# Autodesk Inventor assembly: erp42_2
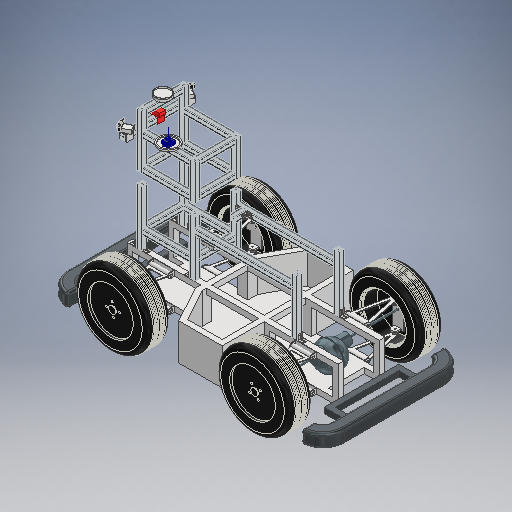
[picture p0: Inventor's stored thumbnail of the model, 512x512]
Saved by Autodesk Inventor 2025.2 (Build 292293000, 293)
## iProperties
Created: 2024-02-06
Part Number: erp42_2
Document SubType Name: Assembly
Designer: ps737
Author: ps737
## Documents named in this file (29)
- C:\Users\jbhma\OneDrive\Desktop\2025_ACCA\2024 ERP42\erp42_2.iam
- C:\Users\jbhma\OneDrive\Desktop\2025_ACCA\2024 ERP42\body.ipt
- C:\Users\jbhma\OneDrive\Desktop\2025_ACCA\2024 ERP42\bumper.ipt
- C:\Users\jbhma\OneDrive\Desktop\2025_ACCA\2024 ERP42\body_braket.ipt
- C:\Users\jbhma\OneDrive\Desktop\2025_ACCA\2024 ERP42\link.ipt
- C:\Users\jbhma\OneDrive\Desktop\2025_ACCA\2024 ERP42\wheel.ipt
- C:\Users\jbhma\OneDrive\Desktop\2025_ACCA\2024 ERP42\wheel_bolt.ipt
- C:\Users\jbhma\OneDrive\Desktop\2025_ACCA\2024 ERP42\프로파일\34.ipt
- C:\Users\jbhma\OneDrive\Desktop\2025_ACCA\2024 ERP42\프로파일\40.5.ipt
- C:\Users\jbhma\OneDrive\Desktop\2025_ACCA\2024 ERP42\L자 브라켓.ipt
- C:\Users\jbhma\OneDrive\Desktop\2025_ACCA\2024 ERP42\wheel_braket_13.ipt
- C:\Users\jbhma\OneDrive\Desktop\2025_ACCA\2024 ERP42\wheel_braket_24.ipt
- C:\Users\jbhma\OneDrive\Desktop\2025_ACCA\2024 ERP42\base_link.ipt
- base_link.ipt
- C:\Users\jbhma\OneDrive\Desktop\2025_ACCA\2024 ERP42\프로파일\8.ipt
- C:\Users\jbhma\OneDrive\Desktop\2025_ACCA\2024 ERP42\프로파일\26.ipt
- C:\Users\jbhma\OneDrive\Desktop\2025_ACCA\2024 ERP42\프로파일\39.ipt
- C:\Users\jbhma\OneDrive\Desktop\2025_ACCA\2024 ERP42\프로파일\70.5.ipt
- C:\Users\jbhma\OneDrive\Desktop\2025_ACCA\2024 ERP42\lidar_case.ipt
- C:\Users\jbhma\OneDrive\Desktop\2025_ACCA\2024 ERP42\86-0138 REV 2, ENVELOPE, VLP-32C M12M.iam
- C:\Users\jbhma\OneDrive\Desktop\2025_ACCA\2024 ERP42\gps_case.ipt
- C:\Users\jbhma\OneDrive\Desktop\2025_ACCA\2024 ERP42\UBLOX_ANN-MB-00_GNSS_ANTENNA.ipt
- C:\Users\jbhma\OneDrive\Desktop\2025_ACCA\2024 ERP42\프로파일\50.ipt
- C:\Users\jbhma\OneDrive\Desktop\2025_ACCA\2024 ERP42\camera_case_front.ipt
- C:\Users\jbhma\OneDrive\Desktop\2025_ACCA\2024 ERP42\camera_case_left.ipt
- C:\Users\jbhma\OneDrive\Desktop\2025_ACCA\2024 ERP42\camera_case_right.ipt
- C:\Users\jbhma\OneDrive\Desktop\2025_ACCA\2024 ERP42\camera.ipt
- C:\Users\jbhma\OneDrive\Desktop\2025_ACCA\2024 ERP42\imu_case.ipt
- C:\Users\jbhma\OneDrive\Desktop\2025_ACCA\2024 ERP42\MTi 600-series STEP files\MTi-600 DEV assembly.iam
## Components (88 placed, 27 different names)
1. body:1 — 메이트:1, 메이트:2, 메이트:3, 메이트:4, 메이트:5, 메이트:6, 메이트:9, 메이트:12, 메이트:60, 메이트:61, 플러쉬:1, 플러쉬:3, 플러쉬:4, 메이트:62, 메이트:64, 메이트:65, 플러쉬:6, 플러쉬:7, 플러쉬:8, 메이트:77, 메이트:78, 메이트:79, 플러쉬:9, 플러쉬:10, 플러쉬:11, 메이트:107, 메이트:108, 플러쉬:21, 플러쉬:22, 메이트:109, 메이트:110, 메이트:124, 플러쉬:28, 각도:18, 플러쉬:29, 각도:19, 플러쉬:31, 플러쉬:32, 플러쉬:33, 메이트:152, 메이트:153, 메이트:154, 각도:20, 각도:21, 각도:22, 각도:23, 메이트:192, 플러쉬:34, 메이트:194, 플러쉬:35, 메이트:196, 플러쉬:36, 메이트:198, 플러쉬:37, 메이트:200, 플러쉬:38, 메이트:202, 플러쉬:39, 메이트:204, 메이트:206, 플러쉬:41, 메이트:209, 플러쉬:42, 메이트:241, 메이트:242, 메이트:243, 플러쉬:60, 메이트:244, 플러쉬:61, 메이트:245, 플러쉬:62, 메이트:252, 메이트:255
2. bumper:1 — 메이트:1, 메이트:2, 플러쉬:6, 플러쉬:10
3. bumper:2 — 메이트:3, 메이트:4, 플러쉬:7, 플러쉬:11, 플러쉬:58
4. body_braket:5 — 메이트:5, 플러쉬:32, 메이트:145, 메이트:151, 메이트:153
5. body_braket:7 — 메이트:6, 메이트:133, 메이트:134, 플러쉬:29, 플러쉬:30
6. body_braket:10 — 메이트:9, 플러쉬:3, 메이트:65, 메이트:144, 메이트:150
7. body_braket:12 — 메이트:12, 플러쉬:1, 메이트:62, 메이트:135, 메이트:136, 플러쉬:30, 플러쉬:40
8. body_braket:15 — 메이트:61, 메이트:140, 메이트:143, 플러쉬:31, 메이트:154
9. body_braket:16 — 메이트:60, 플러쉬:4, 메이트:64, 메이트:141, 메이트:142
10. body_braket:17 — 메이트:79, 플러쉬:33, 메이트:146, 메이트:148, 메이트:152
11. body_braket:18 — 메이트:77, 메이트:78, 플러쉬:9, 메이트:147, 메이트:149
12. 40.5:1 — 메이트:107, 플러쉬:21, 메이트:109, 메이트:201, 메이트:225, 플러쉬:52, 플러쉬:59, 플러쉬:110
13. 40.5:2 — 메이트:108, 플러쉬:22, 메이트:110, 메이트:205, 플러쉬:42, 메이트:224, 플러쉬:51, 플러쉬:109
14. 40.5:3 — 메이트:124, 플러쉬:28, 메이트:203, 메이트:214, 메이트:227, 플러쉬:53, 메이트:249, 플러쉬:66, 메이트:274, 플러쉬:107
15. link:19 — 메이트:129, 메이트:130, 메이트:133, 메이트:134
16. wheel_braket_13:1 — 메이트:131, 메이트:132, 각도:19, 메이트:137, 메이트:139, 메이트:179, 각도:23, 메이트:185
17. wheel_bolt:11 — 메이트:129, 메이트:130, 메이트:131, 메이트:132
18. link:20 — 메이트:135, 메이트:136, 각도:18, 메이트:138, 메이트:240
19. wheel_bolt:12 — 메이트:137, 메이트:138, 메이트:139, 메이트:240
20. link:21 — 메이트:141, 메이트:142, 메이트:175, 메이트:177
21. link:22 — 메이트:140, 메이트:143, 메이트:176, 메이트:178, 메이트:184
22. link:23 — 메이트:146, 메이트:148, 메이트:172, 메이트:174
23. link:24 — 메이트:147, 메이트:149, 메이트:171, 메이트:173
24. link:25 — 메이트:144, 메이트:150, 메이트:167, 메이트:168
25. link:26 — 메이트:145, 메이트:151, 메이트:169, 메이트:170
26. wheel:1 — 메이트:186, 메이트:187
27. wheel:2 — 메이트:179, 메이트:185
28. wheel:3 — 메이트:190, 메이트:191
29. wheel:4 — 메이트:188, 메이트:189, 메이트:208, 메이트:210
30. wheel_braket_13:2 — 메이트:155, 메이트:156, 메이트:161, 메이트:162, 각도:21, 메이트:190, 메이트:191
31. wheel_braket_24:1 — 메이트:180, 메이트:181, 메이트:182, 메이트:183, 각도:20, 메이트:186, 메이트:187
32. wheel_braket_24:2 — 메이트:157, 메이트:158, 메이트:163, 메이트:164, 각도:22, 메이트:188, 메이트:189
33. wheel_bolt:13 — 메이트:158, 메이트:163, 메이트:172, 메이트:174
34. wheel_bolt:14 — 메이트:155, 메이트:161, 메이트:169, 메이트:170
35. wheel_bolt:15 — 메이트:157, 메이트:164, 메이트:171, 메이트:173
36. wheel_bolt:16 — 메이트:156, 메이트:162, 메이트:167, 메이트:168
37. wheel_bolt:17 — 메이트:175, 메이트:177, 메이트:180, 메이트:181, 메이트:183
38. wheel_bolt:18 — 메이트:176, 메이트:178, 메이트:182, 메이트:184
39. L자 브라켓:1 — 메이트:194, 플러쉬:35
40. L자 브라켓:2 — 메이트:192, 플러쉬:34
41. L자 브라켓:3 — 메이트:196, 플러쉬:36
42. L자 브라켓:4 — 메이트:198, 플러쉬:37
43. L자 브라켓:5 — 메이트:202, 메이트:203, 플러쉬:39
44. L자 브라켓:6 — 메이트:200, 메이트:201, 플러쉬:38, 플러쉬:59
45. L자 브라켓:7 — 메이트:204, 메이트:205, 플러쉬:40
46. L자 브라켓:8 — 메이트:206, 플러쉬:41, 메이트:250
47. base_link:1 — 메이트:208, 메이트:209, 메이트:210
48. 8:1 — 메이트:214, 메이트:217, 메이트:218
49. L자 브라켓:9 — 메이트:217
50. L자 브라켓:10 — 메이트:218
51. L자 브라켓:13
52. L자 브라켓:14 — 메이트:224, 플러쉬:51, 메이트:275
53. L자 브라켓:15 — 메이트:225, 플러쉬:52, 메이트:276
54. L자 브라켓:17 — 메이트:227, 플러쉬:53
55. 40.5:4 — 메이트:243, 플러쉬:60, 메이트:246, 플러쉬:64, 메이트:251, 메이트:253, 플러쉬:67, 플러쉬:105, 플러쉬:106
56. 40.5:5 — 메이트:245, 플러쉬:62, 메이트:247, 플러쉬:63, 메이트:254, 플러쉬:68
57. 40.5:6 — 메이트:244, 플러쉬:61, 메이트:248, 플러쉬:65, 메이트:250, 메이트:251, 메이트:252, 메이트:273, 플러쉬:108, 플러쉬:122
58. 26:1 — 메이트:246, 메이트:247, 플러쉬:63, 플러쉬:64, 플러쉬:69, 플러쉬:70, 플러쉬:71, 메이트:255
59. 26:2 — 메이트:248, 메이트:249, 플러쉬:65, 플러쉬:66, 플러쉬:71, 메이트:303, 플러쉬:123
60. 34:1 — 메이트:253, 플러쉬:67, 플러쉬:70
61. 34:2 — 메이트:254, 플러쉬:68, 플러쉬:69
62. 39:3 — 메이트:260, 메이트:262, 플러쉬:72, 플러쉬:75, 플러쉬:76, 플러쉬:86, 메이트:268, 플러쉬:95, 플러쉬:96, 플러쉬:105, 플러쉬:106, 메이트:282
63. 39:4 — 메이트:261, 메이트:263, 플러쉬:73, 플러쉬:74, 플러쉬:77, 플러쉬:87, 메이트:270, 플러쉬:97, 플러쉬:98, 메이트:299, 플러쉬:120
64. 26:3 — 메이트:264, 메이트:267, 플러쉬:92, 플러쉬:93, 플러쉬:94
65. 26:4 — 메이트:260, 메이트:261, 플러쉬:72, 플러쉬:73, 플러쉬:74, 플러쉬:75, 각도:24, 각도:25, 플러쉬:111, 메이트:298
66. 26:5 — 메이트:262, 메이트:263, 플러쉬:76, 플러쉬:77, 플러쉬:86, 플러쉬:87
67. 26:6 — 메이트:265, 플러쉬:88, 플러쉬:89, 플러쉬:90, 플러쉬:91, 플러쉬:119
68. 26:7 — 플러쉬:90, 메이트:267, 플러쉬:91, 플러쉬:93, 플러쉬:99, 플러쉬:100, 메이트:271, 플러쉬:102, 플러쉬:103
69. 26:8 — 메이트:264, 메이트:265, 플러쉬:88, 플러쉬:89, 플러쉬:92, 플러쉬:94, 메이트:269, 메이트:272, 플러쉬:101, 플러쉬:104
70. 34:4 — 메이트:268, 메이트:269, 플러쉬:95, 플러쉬:96
71. 34:5 — 메이트:270, 플러쉬:97, 플러쉬:98, 플러쉬:99, 플러쉬:100
72. 34:6 — 메이트:271, 플러쉬:102, 플러쉬:103, 플러쉬:121
73. 34:7 — 메이트:272, 플러쉬:101, 플러쉬:104, 메이트:285, 플러쉬:112
74. 70.5:2 — 메이트:274, 플러쉬:107, 플러쉬:109, 메이트:276
75. 70.5:3 — 메이트:273, 플러쉬:108, 플러쉬:110, 메이트:275
76. lidar_case:1 — 각도:24, 메이트:280, 메이트:281, 메이트:282, 메이트:298
77. 86-0138 REV 2, ENVELOPE, VLP-32C M12M:1 [sub-assembly] — 메이트:280, 메이트:281, 각도:25, 플러쉬:111
78. gps_case:1 — 메이트:284, 메이트:285, 플러쉬:112
79. UBLOX_ANN-MB-00_GNSS_ANTENNA:1 — 메이트:284, 플러쉬:119
80. 50:1 — 메이트:292, 메이트:293, 메이트:294, 메이트:295, 메이트:296, 메이트:297, 플러쉬:116, 플러쉬:117, 플러쉬:118, 메이트:299, 플러쉬:120, 플러쉬:121
81. camera_case_front:1 — 메이트:290, 메이트:291, 플러쉬:115, 메이트:292, 메이트:293, 플러쉬:116
82. camera_case_left:1 — 메이트:286, 메이트:287, 플러쉬:113, 메이트:294, 메이트:295, 플러쉬:118
83. camera_case_right:1 — 메이트:288, 메이트:289, 플러쉬:114, 메이트:296, 메이트:297, 플러쉬:117
84. camera:1 — 메이트:288, 메이트:289, 플러쉬:114
85. camera:2 — 메이트:286, 메이트:287, 플러쉬:113
86. camera:3 — 메이트:290, 메이트:291, 플러쉬:115
87. imu_case:1 — 메이트:303, 플러쉬:122, 플러쉬:123
88. MTi-600 DEV assembly:1 [sub-assembly]
## Relationships (252: Mate 156, Flush 87, Angle 9)
- 메이트:1 [Mate]: body:1 ↔ bumper:1
- 메이트:2 [Mate]: body:1 ↔ bumper:1
- 메이트:3 [Mate]: body:1 ↔ bumper:2
- 메이트:4 [Mate]: body:1 ↔ bumper:2
- 메이트:5 [Mate]: body:1 ↔ body_braket:5
- 메이트:6 [Mate]: body:1 ↔ body_braket:7
- 메이트:9 [Mate]: body:1 ↔ body_braket:10
- 메이트:12 [Mate]: body:1 ↔ body_braket:12
- 메이트:60 [Mate]: body:1 ↔ body_braket:16
- 메이트:61 [Mate]: body:1 ↔ body_braket:15
- 플러쉬:1 [Flush]: body:1 ↔ body_braket:12
- 플러쉬:3 [Flush]: body:1 ↔ body_braket:10
- 플러쉬:4 [Flush]: body:1 ↔ body_braket:16
- 메이트:62 [Mate] (230 mm): body:1 ↔ body_braket:12
- 메이트:64 [Mate] (190 mm): body:1 ↔ body_braket:16
- 메이트:65 [Mate] (190 mm): body:1 ↔ body_braket:10
- 플러쉬:6 [Flush] (-25 mm): body:1 ↔ bumper:1
- 플러쉬:7 [Flush] (-25 mm): body:1 ↔ bumper:2
- 플러쉬:8 [Flush] (105 mm): body:1
- 메이트:77 [Mate]: body:1 ↔ body_braket:18
- 메이트:78 [Mate] (230 mm): body:1 ↔ body_braket:18
- 메이트:79 [Mate]: body:1 ↔ body_braket:17
- 플러쉬:9 [Flush]: body:1 ↔ body_braket:18
- 플러쉬:10 [Flush] (100 mm): body:1 ↔ bumper:1
- 플러쉬:11 [Flush] (100 mm): body:1 ↔ bumper:2
- 메이트:107 [Mate]: body:1 ↔ 40.5:1
- 메이트:108 [Mate]: body:1 ↔ 40.5:2
- 플러쉬:21 [Flush]: body:1 ↔ 40.5:1
- 플러쉬:22 [Flush]: body:1 ↔ 40.5:2
- 메이트:109 [Mate] (200 mm): body:1 ↔ 40.5:1
- 메이트:110 [Mate] (200 mm): body:1 ↔ 40.5:2
- 메이트:124 [Mate]: body:1 ↔ 40.5:3
- 플러쉬:28 [Flush]: body:1 ↔ 40.5:3
- 메이트:129 [Mate]: link:19 ↔ wheel_bolt:11
- 메이트:130 [Mate]: link:19 ↔ wheel_bolt:11
- 메이트:131 [Mate]: wheel_braket_13:1 ↔ wheel_bolt:11
- 메이트:132 [Mate]: wheel_braket_13:1 ↔ wheel_bolt:11
- 메이트:133 [Mate]: body_braket:7 ↔ link:19
- 메이트:134 [Mate]: body_braket:7 ↔ link:19
- 메이트:135 [Mate]: body_braket:12 ↔ link:20
- 메이트:136 [Mate]: body_braket:12 ↔ link:20
- 각도:18 [Angle] (0 deg): body:1 ↔ link:20
- 플러쉬:29 [Flush]: body:1 ↔ body_braket:7
- 각도:19 [Angle] (180 deg): body:1 ↔ wheel_braket_13:1
- 플러쉬:30 [Flush]: body_braket:7 ↔ body_braket:12
- 메이트:137 [Mate]: wheel_braket_13:1 ↔ wheel_bolt:12
- 메이트:138 [Mate]: link:20 ↔ wheel_bolt:12
- 메이트:139 [Mate]: wheel_braket_13:1 ↔ wheel_bolt:12
- 메이트:140 [Mate]: body_braket:15 ↔ link:22
- 메이트:141 [Mate]: body_braket:16 ↔ link:21
- 메이트:142 [Mate]: body_braket:16 ↔ link:21
- 메이트:143 [Mate]: body_braket:15 ↔ link:22
- 플러쉬:31 [Flush]: body:1 ↔ body_braket:15
- 플러쉬:32 [Flush]: body:1 ↔ body_braket:5
- 플러쉬:33 [Flush]: body:1 ↔ body_braket:17
- 메이트:144 [Mate]: body_braket:10 ↔ link:25
- 메이트:145 [Mate]: body_braket:5 ↔ link:26
- 메이트:146 [Mate]: body_braket:17 ↔ link:23
- 메이트:147 [Mate]: body_braket:18 ↔ link:24
- 메이트:148 [Mate]: body_braket:17 ↔ link:23
- 메이트:149 [Mate]: body_braket:18 ↔ link:24
- 메이트:150 [Mate]: body_braket:10 ↔ link:25
- 메이트:151 [Mate]: body_braket:5 ↔ link:26
- 메이트:152 [Mate] (230 mm): body:1 ↔ body_braket:17
- 메이트:153 [Mate] (190 mm): body:1 ↔ body_braket:5
- 메이트:154 [Mate] (190 mm): body:1 ↔ body_braket:15
- 메이트:155 [Mate]: wheel_braket_13:2 ↔ wheel_bolt:14
- 메이트:156 [Mate]: wheel_braket_13:2 ↔ wheel_bolt:16
- 메이트:157 [Mate]: wheel_braket_24:2 ↔ wheel_bolt:15
- 메이트:158 [Mate]: wheel_braket_24:2 ↔ wheel_bolt:13
- 메이트:161 [Mate]: wheel_braket_13:2 ↔ wheel_bolt:14
- 메이트:162 [Mate]: wheel_braket_13:2 ↔ wheel_bolt:16
- 메이트:163 [Mate]: wheel_braket_24:2 ↔ wheel_bolt:13
- 메이트:164 [Mate]: wheel_braket_24:2 ↔ wheel_bolt:15
- 메이트:167 [Mate]: link:25 ↔ wheel_bolt:16
- 메이트:168 [Mate]: link:25 ↔ wheel_bolt:16
- 메이트:169 [Mate]: link:26 ↔ wheel_bolt:14
- 메이트:170 [Mate]: link:26 ↔ wheel_bolt:14
- 메이트:171 [Mate]: link:24 ↔ wheel_bolt:15
- 메이트:172 [Mate]: link:23 ↔ wheel_bolt:13
- 메이트:173 [Mate]: link:24 ↔ wheel_bolt:15
- 메이트:174 [Mate]: link:23 ↔ wheel_bolt:13
- 메이트:175 [Mate]: link:21 ↔ wheel_bolt:17
- 메이트:176 [Mate]: link:22 ↔ wheel_bolt:18
- 메이트:177 [Mate]: link:21 ↔ wheel_bolt:17
- 메이트:178 [Mate]: link:22 ↔ wheel_bolt:18
- 메이트:179 [Mate]: wheel_braket_13:1 ↔ wheel:2
- 메이트:180 [Mate]: wheel_braket_24:1 ↔ wheel_bolt:17
- 메이트:181 [Mate]: wheel_braket_24:1 ↔ wheel_bolt:17
- 메이트:182 [Mate]: wheel_braket_24:1 ↔ wheel_bolt:18
- 메이트:183 [Mate]: wheel_braket_24:1 ↔ wheel_bolt:17
- 메이트:184 [Mate]: link:22 ↔ wheel_bolt:18
- 각도:20 [Angle] (180 deg): body:1 ↔ wheel_braket_24:1
- 각도:21 [Angle] (180 deg): body:1 ↔ wheel_braket_13:2
- 각도:22 [Angle] (180 deg): body:1 ↔ wheel_braket_24:2
- 각도:23 [Angle] (180 deg): body:1 ↔ wheel_braket_13:1
- 메이트:185 [Mate]: wheel_braket_13:1 ↔ wheel:2
- 메이트:186 [Mate]: wheel:1 ↔ wheel_braket_24:1
- 메이트:187 [Mate]: wheel:1 ↔ wheel_braket_24:1
- 메이트:188 [Mate]: wheel:4 ↔ wheel_braket_24:2
- 메이트:189 [Mate]: wheel:4 ↔ wheel_braket_24:2
- 메이트:190 [Mate]: wheel:3 ↔ wheel_braket_13:2
- 메이트:191 [Mate]: wheel:3 ↔ wheel_braket_13:2
- 메이트:192 [Mate]: body:1 ↔ L자 브라켓:2
- 플러쉬:34 [Flush] (2.5 mm): body:1 ↔ L자 브라켓:2
- 메이트:194 [Mate]: body:1 ↔ L자 브라켓:1
- 플러쉬:35 [Flush] (2.5 mm): body:1 ↔ L자 브라켓:1
- 메이트:196 [Mate]: body:1 ↔ L자 브라켓:3
- 플러쉬:36 [Flush] (2.2 mm): body:1 ↔ L자 브라켓:3
- 메이트:198 [Mate]: body:1 ↔ L자 브라켓:4
- 플러쉬:37 [Flush] (2.5 mm): body:1 ↔ L자 브라켓:4
- 메이트:200 [Mate]: body:1 ↔ L자 브라켓:6
- 메이트:201 [Mate]: 40.5:1 ↔ L자 브라켓:6
- 플러쉬:38 [Flush] (2.5 mm): body:1 ↔ L자 브라켓:6
- 메이트:202 [Mate]: body:1 ↔ L자 브라켓:5
- 메이트:203 [Mate]: 40.5:3 ↔ L자 브라켓:5
- 플러쉬:39 [Flush] (2.5 mm): body:1 ↔ L자 브라켓:5
- 메이트:204 [Mate]: body:1 ↔ L자 브라켓:7
- 메이트:205 [Mate]: 40.5:2 ↔ L자 브라켓:7
- 플러쉬:40 [Flush] (2.5 mm): body_braket:12 ↔ L자 브라켓:7
- 메이트:206 [Mate]: body:1 ↔ L자 브라켓:8
- 플러쉬:41 [Flush] (2.5 mm): body:1 ↔ L자 브라켓:8
- 메이트:208 [Mate]: wheel:4 ↔ base_link:1
- 메이트:209 [Mate]: body:1 ↔ base_link:1
- 메이트:210 [Mate]: wheel:4 ↔ base_link:1
- 플러쉬:42 [Flush]: body:1 ↔ 40.5:2
- 메이트:214 [Mate] (40 mm): 40.5:3 ↔ 8:1
- 메이트:217 [Mate]: 8:1 ↔ L자 브라켓:9
- 메이트:218 [Mate]: 8:1 ↔ L자 브라켓:10
- 메이트:224 [Mate]: 40.5:2 ↔ L자 브라켓:14
- 플러쉬:51 [Flush] (2.5 mm): 40.5:2 ↔ L자 브라켓:14
- 메이트:225 [Mate]: 40.5:1 ↔ L자 브라켓:15
- 플러쉬:52 [Flush] (2.5 mm): 40.5:1 ↔ L자 브라켓:15
- 메이트:227 [Mate]: 40.5:3 ↔ L자 브라켓:17
- 플러쉬:53 [Flush] (2.5 mm): 40.5:3 ↔ L자 브라켓:17
- 메이트:240 [Mate]: link:20 ↔ wheel_bolt:12
- 메이트:241 [Mate] (-170 mm): body:1
- 메이트:242 [Mate] (105 mm): body:1
- 플러쉬:58 [Flush] (-990 mm): bumper:2
- 플러쉬:59 [Flush] (2.5 mm): 40.5:1 ↔ L자 브라켓:6
- 메이트:243 [Mate]: body:1 ↔ 40.5:4
- 플러쉬:60 [Flush]: body:1 ↔ 40.5:4
- 메이트:244 [Mate]: body:1 ↔ 40.5:6
- 플러쉬:61 [Flush]: body:1 ↔ 40.5:6
- 메이트:245 [Mate]: body:1 ↔ 40.5:5
- 플러쉬:62 [Flush]: body:1 ↔ 40.5:5
- 메이트:246 [Mate]: 40.5:4 ↔ 26:1
- 메이트:247 [Mate]: 40.5:5 ↔ 26:1
- 플러쉬:63 [Flush]: 40.5:5 ↔ 26:1
- 플러쉬:64 [Flush]: 40.5:4 ↔ 26:1
- 메이트:248 [Mate]: 40.5:6 ↔ 26:2
- 메이트:249 [Mate]: 40.5:3 ↔ 26:2
- 플러쉬:65 [Flush]: 40.5:6 ↔ 26:2
- 플러쉬:66 [Flush]: 40.5:3 ↔ 26:2
- 메이트:250 [Mate]: L자 브라켓:8 ↔ 40.5:6
- 메이트:251 [Mate] (340 mm): 40.5:4 ↔ 40.5:6
- 메이트:252 [Mate] (45 mm): body:1 ↔ 40.5:6
- 메이트:253 [Mate]: 40.5:4 ↔ 34:1
- 메이트:254 [Mate]: 40.5:5 ↔ 34:2
- 플러쉬:67 [Flush]: 40.5:4 ↔ 34:1
- 플러쉬:68 [Flush]: 40.5:5 ↔ 34:2
- 플러쉬:69 [Flush]: 26:1 ↔ 34:2
- 플러쉬:70 [Flush]: 26:1 ↔ 34:1
- 플러쉬:71 [Flush]: 26:1 ↔ 26:2
- 메이트:255 [Mate] (100 mm): body:1 ↔ 26:1
- 메이트:260 [Mate]: 39:3 ↔ 26:4
- 메이트:261 [Mate]: 39:4 ↔ 26:4
- 메이트:262 [Mate]: 39:3 ↔ 26:5
- 메이트:263 [Mate]: 39:4 ↔ 26:5
- 플러쉬:72 [Flush]: 39:3 ↔ 26:4
- 플러쉬:73 [Flush]: 39:4 ↔ 26:4
- 플러쉬:74 [Flush]: 39:4 ↔ 26:4
- 플러쉬:75 [Flush]: 39:3 ↔ 26:4
- 플러쉬:76 [Flush]: 39:3 ↔ 26:5
- 플러쉬:77 [Flush]: 39:4 ↔ 26:5
- 플러쉬:86 [Flush]: 39:3 ↔ 26:5
- 플러쉬:87 [Flush]: 39:4 ↔ 26:5
- 메이트:264 [Mate]: 26:3 ↔ 26:8
- 메이트:265 [Mate]: 26:6 ↔ 26:8
- 플러쉬:88 [Flush]: 26:6 ↔ 26:8
- 플러쉬:89 [Flush]: 26:6 ↔ 26:8
- 플러쉬:90 [Flush]: 26:6 ↔ 26:7
- 메이트:267 [Mate]: 26:3 ↔ 26:7
- 플러쉬:91 [Flush]: 26:6 ↔ 26:7
- 플러쉬:92 [Flush]: 26:3 ↔ 26:8
- 플러쉬:93 [Flush]: 26:3 ↔ 26:7
- 플러쉬:94 [Flush]: 26:3 ↔ 26:8
- 메이트:268 [Mate]: 39:3 ↔ 34:4
- 메이트:269 [Mate]: 26:8 ↔ 34:4
- 플러쉬:95 [Flush]: 39:3 ↔ 34:4
- 플러쉬:96 [Flush]: 39:3 ↔ 34:4
- 메이트:270 [Mate]: 39:4 ↔ 34:5
- 플러쉬:97 [Flush]: 39:4 ↔ 34:5
- 플러쉬:98 [Flush]: 39:4 ↔ 34:5
- 플러쉬:99 [Flush]: 26:7 ↔ 34:5
- 플러쉬:100 [Flush]: 26:7 ↔ 34:5
- 메이트:271 [Mate]: 26:7 ↔ 34:6
- 메이트:272 [Mate]: 26:8 ↔ 34:7
- 플러쉬:101 [Flush]: 26:8 ↔ 34:7
- 플러쉬:102 [Flush]: 26:7 ↔ 34:6
- 플러쉬:103 [Flush]: 26:7 ↔ 34:6
- 플러쉬:104 [Flush]: 26:8 ↔ 34:7
- 플러쉬:105 [Flush]: 40.5:4 ↔ 39:3
- 플러쉬:106 [Flush]: 40.5:4 ↔ 39:3
- 메이트:273 [Mate]: 40.5:6 ↔ 70.5:3
- 메이트:274 [Mate]: 40.5:3 ↔ 70.5:2
- 플러쉬:107 [Flush]: 40.5:3 ↔ 70.5:2
- 플러쉬:108 [Flush]: 40.5:6 ↔ 70.5:3
- 플러쉬:109 [Flush] (73 mm): 40.5:2 ↔ 70.5:2
- 플러쉬:110 [Flush] (73 mm): 40.5:1 ↔ 70.5:3
- 메이트:275 [Mate]: L자 브라켓:14 ↔ 70.5:3
- 메이트:276 [Mate]: L자 브라켓:15 ↔ 70.5:2
- 각도:24 [Angle] (90 deg): 26:4 ↔ lidar_case:1
- 메이트:280 [Mate]: lidar_case:1 ↔ 86-0138 REV 2, ENVELOPE, VLP-32C M12M:1
- 메이트:281 [Mate]: lidar_case:1 ↔ 86-0138 REV 2, ENVELOPE, VLP-32C M12M:1
- 메이트:282 [Mate] (137 mm): 39:3 ↔ lidar_case:1
- 각도:25 [Angle] (180 deg): 26:4 ↔ 86-0138 REV 2, ENVELOPE, VLP-32C M12M:1
- 플러쉬:111 [Flush] (-39.055 mm): 26:4 ↔ 86-0138 REV 2, ENVELOPE, VLP-32C M12M:1
- [Mate]: gps_case:1 ↔ UBLOX_ANN-MB-00_GNSS_ANTENNA:1
- [Angle] (270 deg): gps_case:1 ↔ UBLOX_ANN-MB-00_GNSS_ANTENNA:1
- 메이트:284 [Mate]: gps_case:1 ↔ UBLOX_ANN-MB-00_GNSS_ANTENNA:1
- 메이트:285 [Mate]: 34:7 ↔ gps_case:1
- 플러쉬:112 [Flush] (25 mm): 34:7 ↔ gps_case:1
- 메이트:286 [Mate]: camera_case_left:1 ↔ camera:2
- 메이트:287 [Mate]: camera_case_left:1 ↔ camera:2
- 플러쉬:113 [Flush] (29 mm): camera_case_left:1 ↔ camera:2
- 메이트:288 [Mate]: camera_case_right:1 ↔ camera:1
- 메이트:289 [Mate]: camera_case_right:1 ↔ camera:1
- 플러쉬:114 [Flush] (29 mm): camera_case_right:1 ↔ camera:1
- 메이트:290 [Mate]: camera_case_front:1 ↔ camera:3
- 메이트:291 [Mate]: camera_case_front:1 ↔ camera:3
- 플러쉬:115 [Flush] (29 mm): camera_case_front:1 ↔ camera:3
- 메이트:292 [Mate]: 50:1 ↔ camera_case_front:1
- 메이트:293 [Mate]: 50:1 ↔ camera_case_front:1
- 메이트:294 [Mate]: 50:1 ↔ camera_case_left:1
- 메이트:295 [Mate]: 50:1 ↔ camera_case_left:1
- 메이트:296 [Mate]: 50:1 ↔ camera_case_right:1
- 메이트:297 [Mate]: 50:1 ↔ camera_case_right:1
- 플러쉬:116 [Flush] (224 mm): 50:1 ↔ camera_case_front:1
- 플러쉬:117 [Flush]: 50:1 ↔ camera_case_right:1
- 플러쉬:118 [Flush]: 50:1 ↔ camera_case_left:1
- 메이트:298 [Mate]: 26:4 ↔ lidar_case:1
- 플러쉬:119 [Flush] (180 mm): 26:6 ↔ UBLOX_ANN-MB-00_GNSS_ANTENNA:1
- 메이트:299 [Mate]: 39:4 ↔ 50:1
- 플러쉬:120 [Flush] (-80 mm): 39:4 ↔ 50:1
- 플러쉬:121 [Flush]: 34:6 ↔ 50:1
- [Mate]: imu_case:1 ↔ MTi-600 DEV assembly:1
- [Mate]: imu_case:1 ↔ MTi-600 DEV assembly:1
- [Mate]: imu_case:1 ↔ MTi-600 DEV assembly:1
- 메이트:303 [Mate]: 26:2 ↔ imu_case:1
- 플러쉬:122 [Flush] (-120.601 mm): 40.5:6 ↔ imu_case:1
- 플러쉬:123 [Flush] (-18.899 mm): 26:2 ↔ imu_case:1
